# Autodesk Inventor assembly: Legstretcher
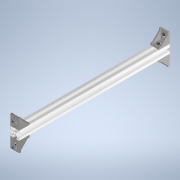
[picture p0: Inventor's stored thumbnail of the model, 180x180]
Saved by Autodesk Inventor 2020.2 (Build 242310000, 310)
## iProperties
Created: 2020-07-25
Part Number: Legstretcher
Document SubType Name: Assembly
Designer: JK
Author: JK
## Documents named in this file (3)
- C:\Users\JK\Documents\Inventor\Mesa\Legstretcher.iam
- C:\Users\JK\Documents\Inventor\Mesa\30x30x500.ipt
- C:\Users\JK\Documents\Inventor\Mesa\Cornerassembly.iam
## Components (5 placed, 2 different names)
1. 30x30x500:1 — Mate:1, Flush:1, Flush:2, Mate:2, Flush:3, Mate:3, Flush:5, Flush:6, Mate:4, Flush:7, Flush:8
2. Cornerassembly:1 [sub-assembly] — Mate:1, Flush:1, Flush:2, Flush:4
3. Cornerassembly:2 [sub-assembly] — Mate:3, Flush:5, Flush:6
4. Cornerassembly:3 [sub-assembly] — Mate:2, Flush:3, Flush:4
5. Cornerassembly:4 [sub-assembly] — Mate:4, Flush:7, Flush:8
## Relationships (12: Flush 8, Mate 4)
- Mate:1: 30x30x500:1 ↔ Cornerassembly:1
- Flush:1: 30x30x500:1 ↔ Cornerassembly:1
- Flush:2 (0.5 mm): 30x30x500:1 ↔ Cornerassembly:1
- Mate:2: 30x30x500:1 ↔ Cornerassembly:3
- Flush:3 (0.5 mm): 30x30x500:1 ↔ Cornerassembly:3
- Flush:4: Cornerassembly:1 ↔ Cornerassembly:3
- Mate:3: 30x30x500:1 ↔ Cornerassembly:2
- Flush:5 (0.5 mm): 30x30x500:1 ↔ Cornerassembly:2
- Flush:6: 30x30x500:1 ↔ Cornerassembly:2
- Mate:4: 30x30x500:1 ↔ Cornerassembly:4
- Flush:7 (0.5 mm): 30x30x500:1 ↔ Cornerassembly:4
- Flush:8: 30x30x500:1 ↔ Cornerassembly:4
